# Autodesk Inventor assembly: M-脚クランク
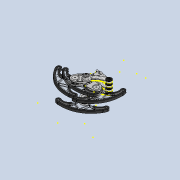
[picture p0: Inventor's stored thumbnail of the model, 180x180]
Saved by Autodesk Inventor 2020 (Build 240168000, 168)
## iProperties
Created: 2021-02-23
Part Number: M-脚クランク
Document SubType Name: Assembly
Designer: AA19065
Mass: 76.8376 g
Surface Area: 596.376 cm^2
Volume: 42.1405 cm^3
Density: 1.82337 g/cm^3
Author: AA19065
## Documents named in this file (3)
- C:\Users\happy\OneDrive\ドキュメント\賢一ファイル\SRDC\試作10-2\アセンブリ\M-脚クランク.iam
- C:\Users\happy\OneDrive\ドキュメント\賢一ファイル\SRDC\試作10-2\アセンブリ\M-ヘッケンv2.iam
- C:\Users\happy\OneDrive\ドキュメント\賢一ファイル\SRDC\試作10-2\アセンブリ\M-脚クランク原動節v2.iam
## Components (5 placed, 2 different names)
1. M-ヘッケンv2:1 [sub-assembly] — 挿入:3, メイト:1
2. M-脚クランク原動節v2:1 [sub-assembly] — 挿入:3, 挿入:4, 挿入:2, 挿入:1
3. M-ヘッケンv2:2 [sub-assembly] — 挿入:4, メイト:2
4. M-ヘッケンv2:3 [sub-assembly] — 挿入:2, メイト:3
5. M-ヘッケンv2:4 [sub-assembly] — 挿入:1, メイト:3, メイト:2, メイト:1
## Relationships (7: Insert 4, Mate 3)
- 挿入:3 [Insert]: M-ヘッケンv2:1 ↔ M-脚クランク原動節v2:1
- 挿入:4 [Insert]: M-脚クランク原動節v2:1 ↔ M-ヘッケンv2:2
- 挿入:2 [Insert]: M-脚クランク原動節v2:1 ↔ M-ヘッケンv2:3
- 挿入:1 [Insert]: M-脚クランク原動節v2:1 ↔ M-ヘッケンv2:4
- メイト:3 [Mate]: M-ヘッケンv2:3 ↔ M-ヘッケンv2:4
- メイト:2 [Mate]: M-ヘッケンv2:2 ↔ M-ヘッケンv2:4
- メイト:1 [Mate]: M-ヘッケンv2:1 ↔ M-ヘッケンv2:4
